# Autodesk Inventor assembly: BGTAB6900VV
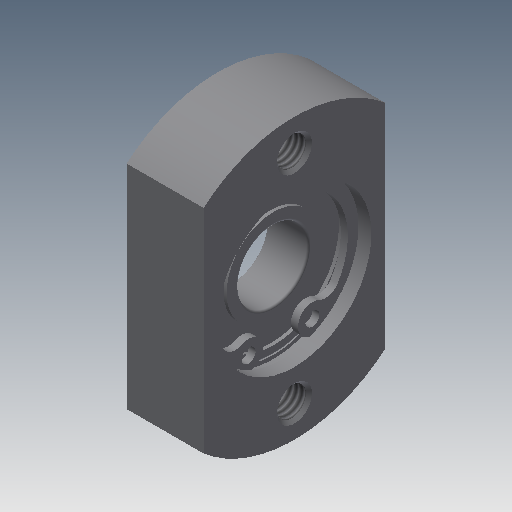
[picture p0: Inventor's stored thumbnail of the model, 512x512]
Saved by Autodesk Inventor 2020.5 (Build 245400000, 400)
## iProperties
Created: 2022-11-21
Part Number: BGTAB6900VV
Catalog Web Link: www.cadenas.de
Description: BGTAB, BGTCA, SBGTA-Bearings with Housings - Space Saving, Small Flange - Retained
Vendor: MISUMI
Document SubType Name: Assembly
Designer: psAdmin
Manufacturer: MISUMI
Mass: 8.03384 g
Surface Area: 53.5072 cm^2
Volume: 8.03384 cm^3
Density: 1 g/cm^3
Category: PARTsolutions
Company: MISUMI
PSOL_IDENT_0: {$CADENAS_DATA/23d-libs/misumi/metric/12_bearing_holders/bgtab_asmtab.prj},206 {VTYP=3D},{STYP=ASSTA
PSOL_IDENT_1: B},{NB=BGTAB6900VV},{LINA=BGTAB6900VV},{NN=BGTAB, BGTCA, SBGTA},{DATE=30.06.2021 12:58:21},{GEOMDATE=
PSOL_IDENT_2: 10.07.2015 02:10:34},{VERSION=},{LINEID=90},{WBVAR=MATB,ST,SEAL,ALT1},{WBNUMERIC=}  {NB=BGTAB6900VV}
PSOL_IDENT_3: ,{LINA=BGTAB6900VV},{KT=DUMMY},{PN=BGTAB6900VV},{TYPE=BGTAB},{MATB=S},{MATBALG= 'S' , 'Steel' , 'SS'
PSOL_IDENT_4: , 'Stainless Steel' },{ST=BO},{STALG= 'BO' , 'Black Oxide' , 'ENP' , 'Electroless Nickel Plating' }
PSOL_IDENT_5: ,{BN=6900},{SEAL=VV},{SEALALG= 'ZZ' , 'Double Shielded' , 'VV' , 'Non-Contact Sealed Rubber Seal' , '
PSOL_IDENT_6: DD' , 'Contact Sealed Rubber Seal' },{DD=10},{D=22},{B=6},{H=40},{W=26},{T=11},{DDHH=19},{A=31},{F=0
PSOL_IDENT_7: },{M=M5},{ALT1=},{M3D=5},{MM=1.15},{BDD2=23},{PPATH=bgtab/bgtab_asmtpl.prj}
NB: BGTAB6900VV
NN: BGTAB, BGTCA, SBGTA
NT: Bearings with Housings - Space Saving, Small Flange - Retained
NBSYN: $PN.
LINA: BGTAB6900VV
CATALOG: Misumi
PN: BGTAB6900VV
MATB: Steel
ST: Black Oxide
BN: 6900
SEAL: Non-Contact Sealed Rubber Seal
DD: 10
D: 22
B: 6
H: 40
W: 26
T: 11
DDHH: 19
A: 31
F: 0
M: M5
ALT1: Bearing and Retaining Ring Assembled
SUPPLIER: MISUMI
ARTICLENO: BGTAB6900VV
BOMINFO: BGTAB6900VV
CREATOR: CADENAS GmbH
Title: BGTAB6900VV
Author: Cadenas PARTsolutions
Comments: Bearings with Housings - Space Saving, Small Flange - Retained
## Documents named in this file (4)
- C:\Users\Administrator\Documents\kamuy2\kamuy2\Parts\BGTAB6900VV_Autodesk_Inventor_2020_20221121\AIS2020\BGTAB6900VV.iam
- C:\Users\Administrator\Documents\kamuy2\kamuy2\Parts\BGTAB6900VV_Autodesk_Inventor_2020_20221121\AIS2020\BGTAB6900VV_h.ipt
- C:\Users\Administrator\Documents\kamuy2\kamuy2\Parts\BGTAB6900VV_Autodesk_Inventor_2020_20221121\AIS2020\bearing_6900.ipt
- C:\Users\Administrator\Documents\kamuy2\kamuy2\Parts\BGTAB6900VV_Autodesk_Inventor_2020_20221121\AIS2020\RRING-C-INT-22.ipt
## Components (3 placed, 3 different names)
1. BGTAB6900VV_h:1 — to_bearings_XY@1 <-> to_housing_XY@2, to_bearings_Z@1 <-> to_housing_Z@2, to_bearings_YZ@1 <-> to_housing_YZ@2, bgcab_to_rring_XY@1 <-> rr_XY@3, bgcab_to_rring_Z@1 <-> rr_Z@3, bgcab_to_rring_YZ@1 <-> rr_YZ@3
2. bearing_6900:1 — to_bearings_XY@1 <-> to_housing_XY@2, to_bearings_Z@1 <-> to_housing_Z@2, to_bearings_YZ@1 <-> to_housing_YZ@2
3. RRING-C-INT-22:1 — bgcab_to_rring_XY@1 <-> rr_XY@3, bgcab_to_rring_Z@1 <-> rr_Z@3, bgcab_to_rring_YZ@1 <-> rr_YZ@3
## Relationships (6: Mate 4, Angle 2)
- to_bearings_XY@1 <-> to_housing_XY@2 [Mate]: BGTAB6900VV_h:1 ↔ bearing_6900:1
- to_bearings_Z@1 <-> to_housing_Z@2 [Mate]: BGTAB6900VV_h:1 ↔ bearing_6900:1
- to_bearings_YZ@1 <-> to_housing_YZ@2 [Angle] (0 deg): BGTAB6900VV_h:1 ↔ bearing_6900:1
- bgcab_to_rring_XY@1 <-> rr_XY@3 [Mate]: BGTAB6900VV_h:1 ↔ RRING-C-INT-22:1
- bgcab_to_rring_Z@1 <-> rr_Z@3 [Mate]: BGTAB6900VV_h:1 ↔ RRING-C-INT-22:1
- bgcab_to_rring_YZ@1 <-> rr_YZ@3 [Angle] (0 deg): BGTAB6900VV_h:1 ↔ RRING-C-INT-22:1
